# Autodesk Inventor assembly: UpperBody
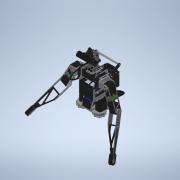
[picture p0: Inventor's stored thumbnail of the model, 180x180]
Saved by Autodesk Inventor 2020 (Build 240168000, 168)
## iProperties
Created: 2016-05-03
Part Number: UpperBody
Document SubType Name: Assembly
Designer: hiroaki
Mass: 2450.59 g
Surface Area: 8110.23 cm^2
Volume: 1381.3 cm^3
Density: 1.77412 g/cm^3
Author: hiroaki
## Documents named in this file (7)
- C:\Users\Masato\Desktop\OpenPlatform_ver3_0 - Ver4_1branch\UpperBody\UpperBody.iam
- C:\Users\Masato\Desktop\OpenPlatform_ver3_0 - Ver4_1branch\UpperBody\Trunk\Trunk.iam
- C:\Users\Masato\Desktop\OpenPlatform_ver3_0 - Ver4_1branch\UpperBody\Head\Head.iam
- C:\Users\Masato\Desktop\OpenPlatform_ver3_0 - Ver4_1branch\UpperBody\Arm\ForeArm.iam
- C:\Users\Masato\Desktop\OpenPlatform_ver3_0 - Ver4_1branch\UpperBody\Arm\Shoulder.iam
- C:\Users\Masato\Desktop\OpenPlatform_ver3_0 - Ver4_1branch\UpperBody\Arm\UpperArm.iam
- C:\Users\Masato\Desktop\OpenPlatform_ver3_0 - Ver4_1branch\UpperBody\Arm\UpperArm_MIR.iam
## Components (8 placed, 6 different names)
1. Head:1 [sub-assembly] — 挿入:13, 角度:12
2. Trunk:1 [sub-assembly] — 挿入:13, 角度:12, 挿入:22, 挿入:23, フラッシュ:10, 角度:24
3. ForeArm:1 [sub-assembly] — 挿入:102, 挿入:103
4. Shoulder:1 [sub-assembly] — 挿入:22, 角度:23, 角度:24, 挿入:100, 挿入:101
5. Shoulder:2 [sub-assembly] — 挿入:23, 角度:23, 挿入:96, 挿入:97
6. UpperArm_MIR:1 [sub-assembly] — 挿入:96, 挿入:97, 挿入:98, 挿入:99
7. ForeArm:2 [sub-assembly] — 挿入:98, 挿入:99
8. UpperArm:1 [sub-assembly] — 挿入:100, 挿入:101, 挿入:102, 挿入:103
## Relationships (15: Insert 11, Angle 3, Flush 1)
- 挿入:13 [Insert]: Head:1 ↔ Trunk:1
- 角度:12 [Angle] (0 deg): Head:1 ↔ Trunk:1
- 挿入:22 [Insert]: Trunk:1 ↔ Shoulder:1
- 挿入:23 [Insert]: Trunk:1 ↔ Shoulder:2
- 角度:23 [Angle] (0 deg): Shoulder:1 ↔ Shoulder:2
- フラッシュ:10 [Flush]: Trunk:1
- 角度:24 [Angle] (0 deg): Trunk:1 ↔ Shoulder:1
- 挿入:96 [Insert]: Shoulder:2 ↔ UpperArm_MIR:1
- 挿入:97 [Insert]: Shoulder:2 ↔ UpperArm_MIR:1
- 挿入:98 [Insert]: UpperArm_MIR:1 ↔ ForeArm:2
- 挿入:99 [Insert]: UpperArm_MIR:1 ↔ ForeArm:2
- 挿入:100 [Insert]: Shoulder:1 ↔ UpperArm:1
- 挿入:101 [Insert]: Shoulder:1 ↔ UpperArm:1
- 挿入:102 [Insert]: ForeArm:1 ↔ UpperArm:1
- 挿入:103 [Insert]: ForeArm:1 ↔ UpperArm:1
